# Autodesk Inventor assembly: 組合3
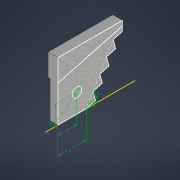
[picture p0: Inventor's stored thumbnail of the model, 180x180]
Saved by Autodesk Inventor 2021 (Build 250183000, 183)
## iProperties
Created: 2020-12-28
Part Number: 組合3
Document SubType Name: Assembly
Designer: zihon
Author: zihon
## Documents named in this file (4)
- C:\Users\zihon\Desktop\組合3.iam
- C:\Users\zihon\Desktop\階梯.ipt
- C:\Users\zihon\Desktop\軸.ipt
- C:\Users\zihon\Desktop\階梯2.ipt
## Components (3 placed, 3 different names)
1. 階梯:1 — 齊平:1, 貼合:4, 齊平:2, 齊平:3, 齊平:4, 貼合:7, 貼合:8
2. 軸:1 — 貼合:4, 貼合:7, 相切:1
3. 階梯2:1 — 貼合:6, 貼合:8, 相切:1
## Relationships (9: Flush 4, Mate 4, Tangent 1)
- 齊平:1 [Flush]: 階梯:1
- 貼合:4 [Mate]: 階梯:1 ↔ 軸:1
- 貼合:6 [Mate]: 階梯2:1
- 齊平:2 [Flush]: 階梯:1
- 齊平:3 [Flush]: 階梯:1
- 齊平:4 [Flush]: 階梯:1
- 貼合:7 [Mate]: 階梯:1 ↔ 軸:1
- 貼合:8 [Mate]: 階梯:1 ↔ 階梯2:1
- 相切:1 [Tangent]: 軸:1 ↔ 階梯2:1
